# Autodesk Inventor assembly: minisumo_złożenie
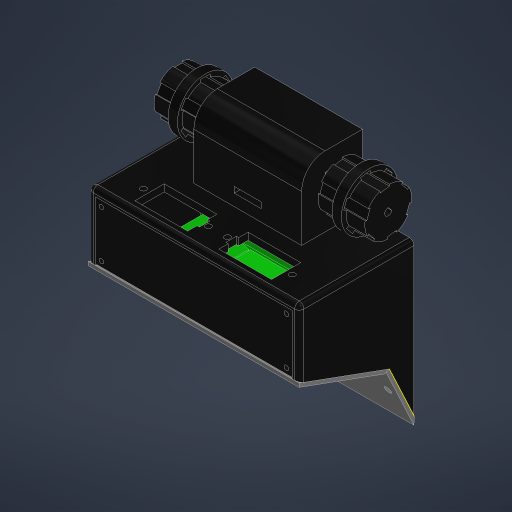
[picture p0: Inventor's stored thumbnail of the model, 512x512]
Saved by Autodesk Inventor 2023.4 (Build 274418000, 418)
## iProperties
Created: 2025-10-31
Part Number: minisumo_złożenie
Document SubType Name: Assembly
Designer: Jakub Borsukiewicz
Author: Jakub Borsukiewicz
## Documents named in this file (7)
- C:\Users\KUBA\Desktop\AiR\Semestr 5\ARES-minisumo-robot\mechanics\minisumo_złożenie.iam
- C:\Users\KUBA\Desktop\AiR\Semestr 5\ARES-minisumo-robot\mechanics\koło.ipt
- C:\Users\KUBA\Desktop\AiR\Semestr 5\ARES-minisumo-robot\mechanics\obudowa_robota.ipt
- C:\Users\KUBA\Desktop\AiR\Semestr 5\ARES-minisumo-robot\mechanics\pług_część1.ipt
- C:\Users\KUBA\Desktop\AiR\Semestr 5\ARES-minisumo-robot\mechanics\pług_część2.ipt
- C:\Users\KUBA\Desktop\AiR\Semestr 5\ARES-minisumo-robot\mechanics\płytka_pcb.ipt
- C:\Users\KUBA\Desktop\AiR\Semestr 5\ARES-minisumo-robot\mechanics\góra_robota.ipt
## Components (7 placed, 6 different names)
1. koło:1 — Obrotowe:1
2. obudowa_robota:1 — Obrotowe:1, Zestawiające:7, Obrotowe:2, Sztywne:1, Sztywne:2, Sztywne:3
3. pług_część1:1 — Sztywne:2
4. pług_część2:1 — Sztywne:3
5. koło:2 — Obrotowe:2
6. płytka_pcb:1 — Zestawiające:7
7. góra_robota:1 — Sztywne:1
## Relationships (6: WeldJoint 3, RevoluteJoint 2, Mate 1)
- Obrotowe:1 [RevoluteJoint] (2 mm): koło:1 ↔ obudowa_robota:1
- Zestawiające:7 [Mate]: obudowa_robota:1 ↔ płytka_pcb:1
- Obrotowe:2 [RevoluteJoint] (2 mm): obudowa_robota:1 ↔ koło:2
- Sztywne:1 [WeldJoint]: obudowa_robota:1 ↔ góra_robota:1
- Sztywne:2 [WeldJoint]: obudowa_robota:1 ↔ pług_część1:1
- Sztywne:3 [WeldJoint]: obudowa_robota:1 ↔ pług_część2:1
